# Autodesk Inventor assembly: case_assambly
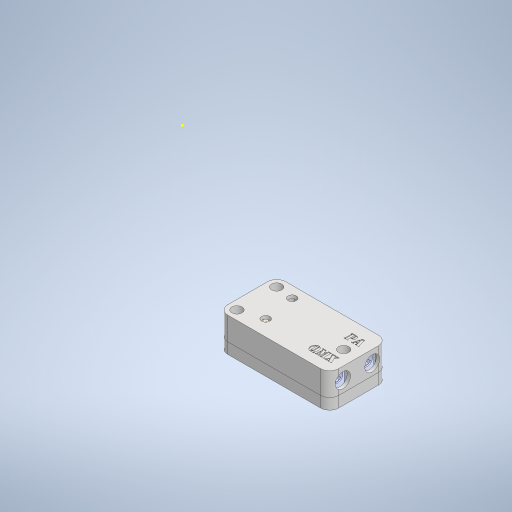
[picture p0: Inventor's stored thumbnail of the model, 512x512]
Saved by Autodesk Inventor 2023 (Build 270158000, 158)
## iProperties
Created: 2024-10-24
Part Number: case_assambly
Document SubType Name: Assembly
Designer: lwerne
Author: lwerne
## Documents named in this file (4)
- C:\Users\lwerne\Nextcloud2\private\HAMpower\Case\case_assambly.iam
- C:\Users\lwerne\Nextcloud2\private\HAMpower\powerplay\powerplay.ipt
- C:\Users\lwerne\Nextcloud2\private\HAMpower\Case\case_base.ipt
- C:\Users\lwerne\Nextcloud2\private\HAMpower\Case\Case_Cap.ipt
## Components (3 placed, 3 different names)
1. powerplay:1 — Flush:1
2. case_base:1 — Flush:1, Flush:2, Flush:3
3. Case_Cap:1 — Flush:2, Flush:3
## Relationships (3: Flush 3)
- Flush:1: powerplay:1 ↔ case_base:1
- Flush:2: case_base:1 ↔ Case_Cap:1
- Flush:3 (10.5 mm): case_base:1 ↔ Case_Cap:1
